# Autodesk Inventor assembly: SAFRS-A-0007
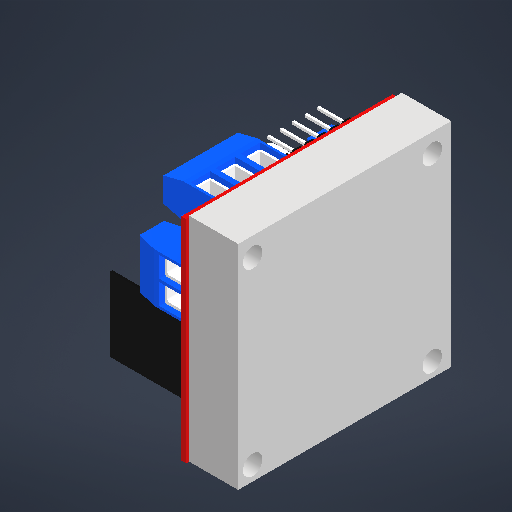
[picture p0: Inventor's stored thumbnail of the model, 512x512]
Saved by Autodesk Inventor 2026.2 (Build 302298000, 298)
## iProperties
Created: 2025-11-26
Part Number: SAFRS-A-0007
Document SubType Name: Assembly
Designer: jaewook
Author: jaewook
Title: L298N Motor Driver Assembly
## Documents named in this file (3)
- C:\Users\jk000\OneDrive\Desktop\git\SAFRS\mechanical\inventor\02__subassemblies\l298n_motor_driver.iam
- C:\Users\jk000\OneDrive\Desktop\git\SAFRS\mechanical\inventor\01_parts\l298n_driver.ipt
- C:\Users\jk000\OneDrive\Desktop\git\SAFRS\mechanical\inventor\01_parts\l298n_base.ipt
## Components (2 placed, 2 different names)
1. l298n_driver:1 — 강체:1
2. l298n_base:1 — 강체:1
## Relationships (1: WeldJoint 1)
- 강체:1 [WeldJoint]: l298n_driver:1 ↔ l298n_base:1
